# Autodesk Inventor assembly: FrontWheelFrameNew
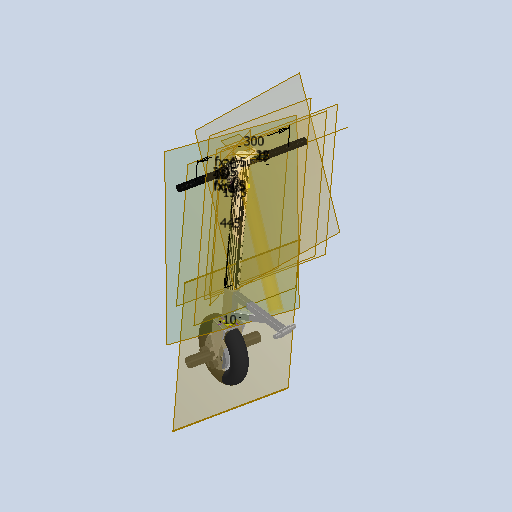
[picture p0: Inventor's stored thumbnail of the model, 512x512]
Saved by Autodesk Inventor 2022.2 (Build 262287000, 287)
## iProperties
Created: 2022-04-06
Part Number: FrontWheelFrameNew
Document SubType Name: Assembly
Designer: Finn Oriwohl
Mass: 3132.3 g
Surface Area: 4455.97 cm^2
Volume: 1821.42 cm^3
Density: 1.7197 g/cm^3
_SolveAssemblyDoc: Frame Generator Solve Assembly
_Version: 25.0.0
Author: Finn Oriwohl
## Documents named in this file (8)
- H:\inventor ting\Mekatronik beercart git\Beercart CAD\Workspaces\Workspace\beercart assembly - mekatronik\Frame\FrontWheelFrameNew.iam
- H:\inventor ting\Mekatronik beercart git\Beercart CAD\Workspaces\Workspace\FrontWheelAssembly.iam
- H:\inventor ting\Mekatronik beercart git\Beercart CAD\Workspaces\Workspace\beercart assembly - mekatronik\Frame\FrontWheelFrameNew\Frame\Frame 1649861603730.iam
- H:\inventor ting\Mekatronik beercart git\Beercart CAD\Workspaces\Workspace\FrontWheelHandle.ipt
- H:\inventor ting\Mekatronik beercart git\Beercart CAD\Workspaces\Workspace\topcap steering handle.ipt
- H:\inventor ting\Mekatronik beercart git\Beercart CAD\Workspaces\Workspace\handelbar screw on extension.ipt
- H:\inventor ting\Mekatronik beercart git\Beercart CAD\Workspaces\Workspace\handelbar side cover.ipt
- H:\inventor ting\Mekatronik beercart git\Beercart CAD\Workspaces\Workspace\frontLightMount.ipt
## Components (8 placed, 7 different names)
1. FrontWheelAssembly:1 [sub-assembly] — Rigid:1, Insert:1
2. FrontWheelMount Frame 1649861603730:1 [sub-assembly] — Insert:1
3. FrontWheelHandle:1 — Rigid:1, Flush:1, Insert:2, Flush:2, Insert:3, Insert:4, Mate:1, Angle:1, Mate:2, Angle:2, Mate:4, Mate:5, Mate:7, Mate:8, Mate:9
4. topcap steering handle:1 — Flush:1, Insert:2
5. handelbar screw on extension:1 — Flush:2, Insert:4
6. handelbar screw on extension:2 — Insert:3, Flush:3, Insert:5
7. handelbar side cover:1 — Flush:3, Insert:5
8. frontLightMount:1 — Flush:4, Mate:8, Mate:9
## Relationships (22: Mate 8, Insert 5, Flush 4, Angle 4, WeldJoint 1)
- Rigid:1 [WeldJoint]: FrontWheelAssembly:1 ↔ FrontWheelHandle:1
- Insert:1 (-18 mm): FrontWheelAssembly:1 ↔ FrontWheelMount Frame 1649861603730:1
- Flush:1: FrontWheelHandle:1 ↔ topcap steering handle:1
- Insert:2: FrontWheelHandle:1 ↔ topcap steering handle:1
- Flush:2: FrontWheelHandle:1 ↔ handelbar screw on extension:1
- Insert:3 (-14 mm): FrontWheelHandle:1 ↔ handelbar screw on extension:2
- Flush:3: handelbar screw on extension:2 ↔ handelbar side cover:1
- Insert:4 (-14 mm): FrontWheelHandle:1 ↔ handelbar screw on extension:1
- Insert:5: handelbar screw on extension:2 ↔ handelbar side cover:1
- Mate:1: FrontWheelHandle:1
- Angle:1 (90 deg): FrontWheelHandle:1
- Mate:2: FrontWheelHandle:1
- Angle:2 (90 deg): FrontWheelHandle:1
- Mate:4: FrontWheelHandle:1
- Mate:5: FrontWheelHandle:1
- Mate:6
- Angle:4 (-15 deg)
- Mate:7: FrontWheelHandle:1
- Angle:5 (0 deg)
- Flush:4: frontLightMount:1
- Mate:8: FrontWheelHandle:1 ↔ frontLightMount:1
- Mate:9: FrontWheelHandle:1 ↔ frontLightMount:1
